# Autodesk Inventor assembly: MotorMount
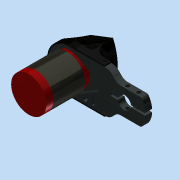
[picture p0: Inventor's stored thumbnail of the model, 180x180]
Saved by Autodesk Inventor 2015 (Build 190159000, 159)
## iProperties
Created: 2015-11-06
Part Number: MotorMount
Document SubType Name: Assembly
Designer: Raphael
Author: Raphael
## Documents named in this file (14)
- \\psf\Home\Documents\electric-skateboard\CAD\MotorMount.iam
- \\psf\Home\Documents\electric-skateboard\CAD\MotorMount.ipt
- \\psf\Home\Documents\electric-skateboard\CAD\Motor.ipt
- \\psf\Home\Documents\electric-skateboard\CAD\18tPulley.ipt
- \\psf\Home\Documents\electric-skateboard\CAD\PulleyCover.ipt
- \\psf\Home\Documents\electric-skateboard\CAD\Encoder.ipt
- \\psf\Home\Documents\electric-skateboard\CAD\M3Bearing.ipt
- \\psf\Home\Documents\electric-skateboard\CAD\Magnet.iam
- \\psf\Home\Documents\electric-skateboard\CAD\MotorMount\AIP\FEA\bliw304tc.fins
- \\psf\Home\Documents\electric-skateboard\CAD\MotorMount\AIP\FEA\bliw304tc.fsat
- \\psf\Home\Documents\electric-skateboard\CAD\MotorMount\AIP\FEA\bliw304tc.ftes
- \\psf\Home\Documents\electric-skateboard\CAD\MotorMount\AIP\FEA\bliw304tc.fwiz
- \\psf\Home\Documents\electric-skateboard\CAD\MotorMount\AIP\FEA\bliw304yo.fmsh
- \\psf\Home\Documents\electric-skateboard\CAD\MotorMount\AIP\FEA\bliw304yp.fres
## Components (8 placed, 7 different names)
1. MotorMount:1 — Mate:1, Mate:2, Mate:4, Mate:5, Flush:1, Mate:9, Mate:10
2. Motor:1 — Mate:1, Mate:2, Mate:3, Mate:14
3. 18tPulley:1 — Mate:3, Mate:13
4. PulleyCover:1 — Mate:4, Mate:5, Flush:1, Mate:6, Mate:7, Mate:8
5. Encoder:1 — Mate:6, Mate:7, Mate:8
6. M3Bearing:1 — Mate:9, Mate:10, Mate:11, Mate:12
7. M3Bearing:2 — Mate:11, Mate:12
8. Magnet:1 [sub-assembly] — Mate:13, Mate:14
## Relationships (15: Mate 14, Flush 1)
- Mate:1: MotorMount:1 ↔ Motor:1
- Mate:2: MotorMount:1 ↔ Motor:1
- Mate:3: Motor:1 ↔ 18tPulley:1
- Mate:4: MotorMount:1 ↔ PulleyCover:1
- Mate:5: MotorMount:1 ↔ PulleyCover:1
- Flush:1: MotorMount:1 ↔ PulleyCover:1
- Mate:6: PulleyCover:1 ↔ Encoder:1
- Mate:7: PulleyCover:1 ↔ Encoder:1
- Mate:8: PulleyCover:1 ↔ Encoder:1
- Mate:9: MotorMount:1 ↔ M3Bearing:1
- Mate:10 (0.5 mm): MotorMount:1 ↔ M3Bearing:1
- Mate:11: M3Bearing:1 ↔ M3Bearing:2
- Mate:12: M3Bearing:1 ↔ M3Bearing:2
- Mate:13: 18tPulley:1 ↔ Magnet:1
- Mate:14: Motor:1 ↔ Magnet:1
## Named parameters: sa_0 = 1955.89, sa_1 = 22154.9, sa_2 = 8.89644e-13
note: some values were not read from the file. Shown as the stored number, unit unknown: "sa_0", "sa_1", "sa_2".
